# Autodesk Inventor assembly: Closing Mechanism Thumbscrew Side
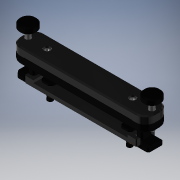
[picture p0: Inventor's stored thumbnail of the model, 180x180]
Saved by Autodesk Inventor 2019 (Build 230136000, 136)
## iProperties
Created: 2018-04-23
Part Number: Closing Mechanism Thumbscrew Side
Document SubType Name: Assembly
Designer: IEUser
Mass: 524.332 g
Surface Area: 910.129 cm^2
Volume: 192.294 cm^3
Density: 2.72672 g/cm^3
Author: IEUser
## Documents named in this file (16)
- C:\Users\IEUser\Desktop\lrut-inflatable-ring-standard-master\Closing Mechanism\Closing Mechanism Thumbscrew Side.iam
- C:\Users\IEUser\Desktop\lrut-inflatable-ring-standard-master\Closing Mechanism\Hard Plate.ipt
- C:\Users\IEUser\Desktop\lrut-inflatable-ring-standard-master\Closing Mechanism\Rail.ipt
- C:\Users\IEUser\Desktop\lrut-inflatable-ring-standard-master\Stock Components\Accu Group\SSCF-M5-16-A4.ipt
- C:\Users\IEUser\Desktop\lrut-inflatable-ring-standard-master\Closing Mechanism\Large Clamp.ipt
- C:\Users\IEUser\Desktop\lrut-inflatable-ring-standard-master\Closing Mechanism\Small Clamp.ipt
- C:\Users\IEUser\Desktop\lrut-inflatable-ring-standard-master\Stock Components\Accu Group\SSK-M5-12-A4.ipt
- C:\Users\IEUser\Desktop\lrut-inflatable-ring-standard-master\Stock Components\Accu Group\SSK-M5-18-A4.ipt
- C:\Users\IEUser\Desktop\lrut-inflatable-ring-standard-master\Closing Mechanism\Top Cover.ipt
- C:\Users\IEUser\Desktop\lrut-inflatable-ring-standard-master\Stock Components\Accu Group\SSCF-M5-10-A4.ipt
- C:\Users\IEUser\Desktop\lrut-inflatable-ring-standard-master\Closing Mechanism\Spigot Plate.ipt
- C:\Users\IEUser\Desktop\lrut-inflatable-ring-standard-master\Spigots\Spigot Short.ipt
- C:\Users\IEUser\Desktop\lrut-inflatable-ring-standard-master\Stock Components\Accu Group\HPCW-M10-A4.ipt
- C:\Users\IEUser\Desktop\lrut-inflatable-ring-standard-master\Stock Components\Elma Electronic\4024-86.ipt
- C:\Users\IEUser\Desktop\lrut-inflatable-ring-standard-master\Stock Components\Amphenol\252124.ipt
- C:\Users\IEUser\Desktop\lrut-inflatable-ring-standard-master\Stock Components\Automotion Components\P0480.080-040-A4.ipt
## Components (31 placed, 15 different names)
1. Hard Plate:1 — Mate:11, Mate:12, Mate:13, Mate:14, Mate:15, Mate:16, Insert:3, Insert:4, Insert:5, Insert:6, Mate:17, Mate:18, Mate:19, Mate:20, Mate:21, Mate:22, Mate:29, Mate:30, Mate:31
2. Rail:1 — Mate:11, Mate:12, Mate:13
3. Rail:2 — Mate:14, Mate:15, Mate:16, Mate:26, Mate:27, Mate:28
4. SSCF-M5-16-A4:1 — Insert:3
5. SSCF-M5-16-A4:2 — Insert:4
6. SSCF-M5-16-A4:3 — Insert:5
7. SSCF-M5-16-A4:4 — Insert:6
8. Large Clamp:1 — Mate:17, Mate:18, Mate:19, Insert:10, Insert:11, Insert:12, Insert:13, Insert:14
9. Small Clamp:1 — Mate:20, Mate:21, Mate:22, Insert:7, Insert:8, Insert:9
10. SSK-M5-12-A4:1 — Insert:7
11. SSK-M5-12-A4:2 — Insert:8
12. SSK-M5-12-A4:3 — Insert:9
13. SSK-M5-18-A4:1 — Insert:10
14. SSK-M5-18-A4:2 — Insert:11
15. SSK-M5-18-A4:3 — Insert:12
16. SSK-M5-18-A4:4 — Insert:13
17. SSK-M5-18-A4:5 — Insert:14
18. Spigot Plate:1 — Mate:26, Mate:27, Mate:28, Insert:17, Angle:1, Insert:18, Angle:2, Insert:19, Insert:20
19. Spigot Short:1 — Insert:17, Angle:1, Insert:23
20. Spigot Short:2 — Insert:18, Angle:2, Insert:24
21. HPCW-M10-A4:1 — Insert:19, Insert:21
22. HPCW-M10-A4:2 — Insert:20, Insert:22
23. 4024-86:1 — Insert:21
24. 4024-86:2 — Insert:22
25. 252124:1 — Insert:23
26. 252124:2 — Insert:24
27. Top Cover:1 — Mate:29, Mate:30, Mate:31, Insert:25, Insert:26, Insert:27, Insert:28
28. SSCF-M5-10-A4:1 — Insert:25
29. SSCF-M5-10-A4:2 — Insert:26
30. P0480.080-040-A4:1 — Insert:27
31. P0480.080-040-A4:2 — Insert:28
## Relationships (44: Insert 24, Mate 18, Angle 2)
- Mate:11: Hard Plate:1 ↔ Rail:1
- Mate:12: Hard Plate:1 ↔ Rail:1
- Mate:13: Hard Plate:1 ↔ Rail:1
- Mate:14: Hard Plate:1 ↔ Rail:2
- Mate:15: Hard Plate:1 ↔ Rail:2
- Mate:16: Hard Plate:1 ↔ Rail:2
- Insert:3: Hard Plate:1 ↔ SSCF-M5-16-A4:1
- Insert:4: Hard Plate:1 ↔ SSCF-M5-16-A4:2
- Insert:5: Hard Plate:1 ↔ SSCF-M5-16-A4:3
- Insert:6: Hard Plate:1 ↔ SSCF-M5-16-A4:4
- Mate:17: Hard Plate:1 ↔ Large Clamp:1
- Mate:18: Hard Plate:1 ↔ Large Clamp:1
- Mate:19: Hard Plate:1 ↔ Large Clamp:1
- Mate:20: Hard Plate:1 ↔ Small Clamp:1
- Mate:21: Hard Plate:1 ↔ Small Clamp:1
- Mate:22: Hard Plate:1 ↔ Small Clamp:1
- Insert:7: Small Clamp:1 ↔ SSK-M5-12-A4:1
- Insert:8: Small Clamp:1 ↔ SSK-M5-12-A4:2
- Insert:9: Small Clamp:1 ↔ SSK-M5-12-A4:3
- Insert:10: Large Clamp:1 ↔ SSK-M5-18-A4:1
- Insert:11: Large Clamp:1 ↔ SSK-M5-18-A4:2
- Insert:12: Large Clamp:1 ↔ SSK-M5-18-A4:3
- Insert:13: Large Clamp:1 ↔ SSK-M5-18-A4:4
- Insert:14: Large Clamp:1 ↔ SSK-M5-18-A4:5
- Mate:26: Rail:2 ↔ Spigot Plate:1
- Mate:27 (1 mm): Rail:2 ↔ Spigot Plate:1
- Mate:28 (0.25 mm): Rail:2 ↔ Spigot Plate:1
- Insert:17 (1 mm): Spigot Plate:1 ↔ Spigot Short:1
- Angle:1 (0 deg): Spigot Plate:1 ↔ Spigot Short:1
- Insert:18 (1 mm): Spigot Plate:1 ↔ Spigot Short:2
- Angle:2 (0 deg): Spigot Plate:1 ↔ Spigot Short:2
- Insert:19 (1 mm): Spigot Plate:1 ↔ HPCW-M10-A4:1
- Insert:20 (1 mm): Spigot Plate:1 ↔ HPCW-M10-A4:2
- Insert:21: HPCW-M10-A4:1 ↔ 4024-86:1
- Insert:22: HPCW-M10-A4:2 ↔ 4024-86:2
- Insert:23: Spigot Short:1 ↔ 252124:1
- Insert:24: Spigot Short:2 ↔ 252124:2
- Mate:29: Hard Plate:1 ↔ Top Cover:1
- Mate:30: Hard Plate:1 ↔ Top Cover:1
- Mate:31: Hard Plate:1 ↔ Top Cover:1
- Insert:25: Top Cover:1 ↔ SSCF-M5-10-A4:1
- Insert:26: Top Cover:1 ↔ SSCF-M5-10-A4:2
- Insert:27 (10 mm): Top Cover:1 ↔ P0480.080-040-A4:1
- Insert:28 (10 mm): Top Cover:1 ↔ P0480.080-040-A4:2
